# Autodesk Inventor assembly: NC_nhk9
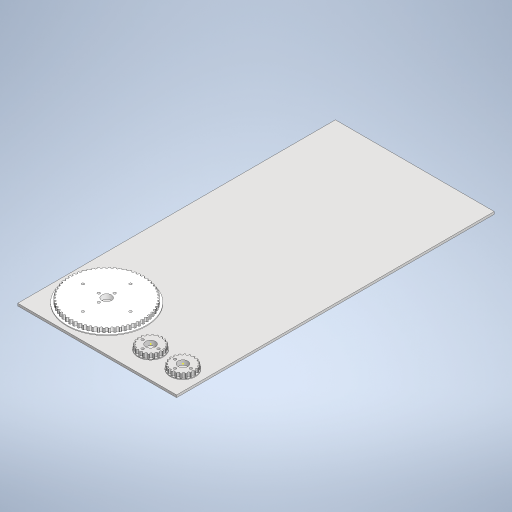
[picture p0: Inventor's stored thumbnail of the model, 512x512]
Saved by Autodesk Inventor 2023 (Build 270158000, 158)
## iProperties
Created: 2022-04-22
Part Number: NC_nhk9
Document SubType Name: Assembly
Designer: yuta
Author: yuta
## Documents named in this file (4)
- C:\Users\yuta\Documents\NHK\NC_nhk9.iam
- C:\Users\yuta\Documents\NHK\NC.port.ipt
- C:\Users\yuta\Documents\NHK\射出_プーリ_歯数60.ipt
- C:\Users\yuta\Documents\NHK\射出_プーリ_歯数20.ipt
## Components (4 placed, 3 different names)
1. NC.port:1 — メイト:1, メイト:2, メイト:3, メイト:4, メイト:5, メイト:6
2. 射出_プーリ_歯数60:1 — メイト:1, メイト:2, メイト:3
3. 射出_プーリ_歯数20:1 — メイト:4
4. 射出_プーリ_歯数20:2 — メイト:5, メイト:6
## Relationships (6: Mate 6)
- メイト:1 [Mate]: NC.port:1 ↔ 射出_プーリ_歯数60:1
- メイト:2 [Mate] (-56 mm): NC.port:1 ↔ 射出_プーリ_歯数60:1
- メイト:3 [Mate] (-56 mm): NC.port:1 ↔ 射出_プーリ_歯数60:1
- メイト:4 [Mate]: NC.port:1 ↔ 射出_プーリ_歯数20:1
- メイト:5 [Mate]: NC.port:1 ↔ 射出_プーリ_歯数20:2
- メイト:6 [Mate] (-24 mm): NC.port:1 ↔ 射出_プーリ_歯数20:2
